# Autodesk Inventor assembly: HTPA32S2M100-A-P5
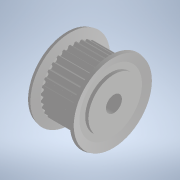
[picture p0: Inventor's stored thumbnail of the model, 180x180]
Saved by Autodesk Inventor 2021 (Build 250183000, 183)
## iProperties
Category: PARTsolutions
Company: MISUMI
Created: 2025-06-07
Part Number: HTPA32S2M100-A-P5
Catalog Web Link: www.cadenas.de
Description: HTPA_ _S2M040, HTPA_ _S2M060, HTPA_ _S2M100, HTPB_ _S2M040, HTPB_ _S2M060, HTPB_ _S2M100, HTPK_ _S2M040, HTPK_ _S2M060, HTPK_ _S2M100, HTPN_ _S2M040, HTPN_ _S2M060, HTPN_ _S2M100, HTPT_ _S2M040, HTPT_ _S2M060, HTPM_ _S2M040, HTPM_ _S2M060, HTPP_ _S2M040, HTPP_ _S2M060, HTPS_ _S2M040, HTPS_ _S2M060, HTPS_ _S2M100-High Torque Timing Pulleys S2M Type
Vendor: MISUMI
Document SubType Name: Assembly
Designer: psAdmin
Manufacturer: MISUMI
Mass: 4.1898 g
Surface Area: 29.6622 cm^2
Volume: 4.1898 cm^3
Density: 1 g/cm^3
Title: HTPA32S2M100-A-P5
Author: Cadenas PARTsolutions
Comments: High Torque Timing Pulleys S2M Type
PSOL_IDENT_0: {$CADENAS_DATA/23d-libs/misumi/metric/51_timing_pulleys/htpm_s2m_asmtab.prj},745 {VTYP=3D},{STYP=ASS
PSOL_IDENT_1: TAB},{NB=HTPA32S2M100-A-P5},{LINA=HTPA32S2M100-A-P5},{NN=HTPA_ _S2M040, HTPA_ _S2M060, HTPA_ _S2M100
PSOL_IDENT_2: , HTPB_ _S2M040, HTPB_ _S2M060, HTPB_ _S2M100, HTPK_ _S2M040, HTPK_ _S2M060, HTPK_ _S2M100, HTPN_ _S
PSOL_IDENT_3: 2M040, HTPN_ _S2M060, HTPN_ _S2M100, HTPT_ _S2M040, HTPT_ _S2M060, HTPM_ _S2M040, HTPM_ _S2M060, HTP
PSOL_IDENT_4: P_ _S2M040, HTPP_ _S2M060, HTPS_ _S2M040, HTPS_ _S2M060, HTPS_ _S2M100},{DATE=13.01.2023 00:39:47},{
PSOL_IDENT_5: GEOMDATE=09.12.2022 07:33:44},{VERSION=},{LINEID=170},{WBVAR=MATP,ST,TNW,PS,SBS,DD,Z,J,Q,R,S,T,ALT1,
PSOL_IDENT_6: ALT2,M,QSC,QFC,QTC,ALT3,K,KSC,KFC,KTC,ALT4,ZM,ZSC,ZFC,ZTC,ALT5,ALT6,ALT7,FC,ALT8,SRG,ALT9,BTC,TL,ALT
PSOL_IDENT_7: 10,TPC,ALT11,BC,ALT12,SLH,ALT13,BN},{WBNUMERIC=DD,Z,J,Q,R,S,T,QSC,QFC,QTC,K,KSC,KFC,KTC,ZSC,ZFC,ZTC,
PSOL_IDENT_8: FC,SRG,BTC,TL,BC,SLH,BN}  {NB=HTPA32S2M100-A-P5},{LINA=HTPA32S2M100-A-P5},{KT=DUMMY},{PN=HTPA32S2M10
PSOL_IDENT_9: 0-A-P5},{TYPE=HTPA},{MATP=A2017},{MATPALG= 'A2017','Aluminum Alloy 2000 series','S45CE','1045 Carbon
PSOL_IDENT_10: Steel Equivalent','SUS304','304 Stainless Steel' },{ST=CA},{STALG= 'CA' , 'Clear Anodize', 'BA','Bl
PSOL_IDENT_11: ack Anodize','HAT','Hard Clear Anodize' , 'ENP' , 'Electroless Nickel Plating' },{NT=32},{TNW=S2M100
PSOL_IDENT_12: },{TNWALG= 'S2M040', 'S2M060','S2M100' },{BW=10},{PS=A},{PSALG='A','B'},{SBS=P},{SBSALG= 'H','Round
PSOL_IDENT_13: Hole','P','Round Hole + Tap','N','New JIS Keywayed Bore + Tap (Standard)','V','Stepped Hole','Y','Bo
PSOL_IDENT_14: th Ends Stepped Hole','WB','Double Stepped Hole' },{SHSA= 'H','Round Hole','P','Round Hole + Tap','N'
PSOL_IDENT_15: ,'New JIS Keywayed Bore + Tap (Standard)','V','Stepped Hole','Y','Both Ends Stepped Hole','WB','Doub
PSOL_IDENT_16: le Stepped Hole' },{SHSB='H','Round Hole','P','Round Hole + Tap','V','Stepped Hole','F','Stepped Hol
PSOL_IDENT_17: e (Counterbore holes on the boss side)' },{SHSK='H','Round Hole','P','Round Hole + Tap'},{SBSPN=-P5}
PSOL_IDENT_18: ,{DD=5.00},{DDALG=[4:4/1],4.5,[5:6/1],6.35,[7:10/1]},{DDHA=[4:4/1],4.5,[5:6/1],6.35,[7:12/1]},{DDHBK=
PSOL_IDENT_19: 0},{DDPA=[4:4/1],4.5,[5:6/1],6.35,[7:10/1]},{DDPBK=0},{DDNA=[8:8/1]},{DDNBK=0},{DDNK=0},{DDCA=0},{DD
PSOL_IDENT_20: CBK=0},{DDVA=[4:4/1],4.5,[5:6/1],6.35,[7:10/1]},{DDVF=0},{DDY=[4:10/1]},{DDWB=[4:8/1]},{Z=0},{ZALG=[
PSOL_IDENT_21: 0]},{ZQRMIN=7},{ZAMAX=12},{ZBMAX=0},{DDZ=5},{J=0.0},{JALG=[0]},{JMAX=13},{JMIN=2},{JPN=},{QRMAX=12},
PSOL_IDENT_22: {QRMIN=7},{WBRMAX=-2.00},{WBQMIN=9},{Q=0},{QALG=[0]},{QPN=},{R=0},{RALG=[0]},{S=0.0},{SALG=[0]},{SPN=
PSOL_IDENT_23: },{SMAX=9},{T=0.0},{TALG=[0]},{TPN=},{TMAX=12},{A=11},{W=15},{L=0},{PD=20.37},{OD=19.86},{D=0},{DALG=
PSOL_IDENT_24: 12},{DE=16},{F=25},{E=16},{BBK=0.000},{TTK=0.0},{TT=1},{WL=15.000},{ALT1=},{ALT1ALG= '','w/o KC90 (S
PSOL_IDENT_25: et Screw Angle)','KC90','with KC90 (Set Screw Angle)' },{ANG=123.750},{ALT1PN=},{ALT2=},{ALT2ALG= ''
PSOL_IDENT_26: ,'Not applicable' },{M=N/A},{MALG= 'N/A' },{MFTALG= 'N/A' },{MSALG= 'N/A' },{M3D=0.000},{KDML=0},{ML=
PSOL_IDENT_27: 0},{MUL=0},{PITCH=0},{QSC=0.0},{QSCALG=0},{QFC=0.0},{QFCALG=0},{QTC=0.0},{QTCALG=0},{QPCDMIN=0},{QPC
PSOL_IDENT_28: DMINALG=0},{QPCDMAX=12},{ALT2PN=},{ALT3=},{ALT3ALG= '','Not applicable' },{K=0.0},{KALG=0},{KMIN=4},
PSOL_IDENT_29: {KFTMAX=0.0},{KSMAX=0.0},{KSC=0.0},{KSCALG=0},{KFC=0.0},{KFCALG=0},{KTC=0.0},{KTCALG=0},{KPCDMIN=9},
PSOL_IDENT_30: {KPCDMINALG=9},{KPCDMAX=12},{KSCMIN=9.0},{KSCMINALG=9},{ALT3PN=},{ALT4=},{ALT4ALG= '','Not applicabl
PSOL_IDENT_31: e' },{ALT4MIN=15.5},{ALT4MAX=5.5},{ZM=N/A},{ZMALG= 'N/A' },{ZMSALG= 'N/A' },{ZMFTALG= 'N/A' },{ZMDD1=
PSOL_IDENT_32: 0.0},{ZMDD2=0.0},{ZMHH=0.0},{ZSC=0.0},{ZSCALG=[0]},{ZFC=0.0},{ZFCALG=[0]},{ZTC=0.0},{ZTCALG=[0]},{ZP
PSOL_IDENT_33: CDMIN=0},{ZPCDMINALG=0},{ZPCDMAX=12},{ALT4PN=},{ALT5=},{ALT5ALG= '','Flange Attached','NFC','with NF
PSOL_IDENT_34: C (Flange not Attached)' },{ALT5PN=},{ALT6=},{ALT6ALG= '','w/o Flange Attached on One Side Only','RF
PSOL_IDENT_35: C','with RFC (Flange Attached on The Boss Side Only)','LFC','with LFC (Flange Attached on The Opposi
PSOL_IDENT_36: te Side Only)' },{ALT6PN=},{ALT7=},{ALT7ALG= '','w/o FC (Flange Cut)','FC','with FC (Flange Cut)' },
PSOL_IDENT_37: {FC=0.0},{FCALG=0},{FCMIN=21.0},{FCMAX=23.0},{ALT7PN=},{ALT8=},{ALT8ALG= '','Not applicable' },{ALT8
PSOL_IDENT_38: ALGALG=12},{ALT8DD2=0},{ALT8MM=0},{ALT8NN=0},{QC=0},{KC=0},{ZC=0},{SRG=0.0},{SRGALG=[0]},{SRGMAX=0},
PSOL_IDENT_39: {DD2=0.0},{MM=0.00},{NN=0.00},{ALT8PN=},{ALT9ALG= '','w/o BTC (Taper for Bearing Holder)','BTC','wit
PSOL_IDENT_40: h BTC (Taper for Bearing Holder)' },{ALT9=},{BTC9=7},{TL9=1},{BTC=0},{BTCALG=[0]},{TL=0.0},{TLALG=[0
PSOL_IDENT_41: ]},{TLMIN=1.000},{TLMAX=-15.500},{BTCL=0},{BTCD=0},{BTCDALG=12.000},{ALT9PN=},{WLBCTL=15},{ALT10=},{
PSOL_IDENT_42: ALT10ALG= '','w/o TPC (Tapped Hole Dimension)','TPC','with TPC (Tapped Hole Dimension)' },{TPC=N/A},
PSOL_IDENT_43: {TPCALG= 'N/A' },{TPCM=3},{ALT10PN=},{ALT11=},{ALT11ALG= '','Not applicable' },{BC=0.0},{BCALG=0},{B
PSOL_IDENT_44: CMIN=6},{BCMAX=-15.5},{BCPLANE=7.5},{M1WBC=7.5},{ALT11PN=},{ALT12=},{ALT12ALG= '','w/o SLH (Set Scre
PSOL_IDENT_45: w Length)','SLH','with SLH (Set Screw Length)' },{SLH=0},{SLHALG=[0]},{ALT12PN=},{ALT13=},{ALT13ALG=
PSOL_IDENT_46: '', 'Not applicable' },{BN=0.0},{BNALG=0},{BNMIN=-14.5},{BNMAX=-5},{ALT13PN=},{AC=M3x3},{M1=3},{M1L=
PSOL_IDENT_47: 3},{TAP=0.000},{KYY=2.5},{KTT=7.43},{PLANE=15},{PPATH=htpm_s2m/htpa_s2m_asmtpl.prj}
NB: HTPA32S2M100-A-P5
NN: 0
NT: 32
NBSYN: $PN.
LINA: HTPA32S2M100-A-P5
CATALOG: Misumi
PN: HTPA32S2M100-A-P5
MATP: Aluminum Alloy 2000 series
ST: Clear Anodize
TNW: S2M100
BW: 10
PS: A
SBS: Round Hole + Tap
DD: 5
Z: 0
J: 0
Q: 0
R: 0
S: 0
T: 0
A: 11
W: 15
L: 0
PD: 20.37
OD: 19.86
D: 0
F: 25
E: 16
TT: 1
ALT1: w/o KC90 (Set Screw Angle)
ALT2: Not applicable
M: N/A
QSC: 0
QFC: 0
QTC: 0
ALT3: Not applicable
K: 0
KSC: 0
KFC: 0
KTC: 0
ALT4: Not applicable
ZM: N/A
ZMDD1: 0
ZMDD2: 0
ZMHH: 0
ZSC: 0
ZFC: 0
ZTC: 0
ALT5: Flange Attached
ALT6: w/o Flange Attached on One Side Only
ALT7: w/o FC (Flange Cut)
FC: 0
ALT8: Not applicable
SRG: 0
DD2: 0
MM: 0
ALT9: w/o BTC (Taper for Bearing Holder)
BTC: 0
TL: 0
BTCL: 0
BTCD: 0
ALT10: w/o TPC (Tapped Hole Dimension)
TPC: N/A
ALT11: Not applicable
BC: 0
ALT12: w/o SLH (Set Screw Length)
SLH: 0
ALT13: Not applicable
BN: 0
AC: M3x3
SUPPLIER: MISUMI
ARTICLENO: HTPA32S2M100-A-P5
BOMINFO: HTPA32S2M100-A-P5
CREATOR: CADENAS GmbH
## Documents named in this file (3)
- e:\temp\worker_COMMON_293\temp\tmp_7720_2_IlNwC\format_0\HTPA32S2M100-A-P5.iam
- e:\temp\worker_COMMON_293\temp\tmp_7720_2_IlNwC\format_0\HTPA32S2M100-A-P5_a.ipt
- e:\temp\worker_COMMON_293\temp\tmp_7720_2_IlNwC\format_0\SET-SCREW3-3.ipt
## Components (3 placed, 2 different names)
1. HTPA32S2M100-A-P5_a:1 — to_s1_Z@1 <-> CP_Z@2, to_s2_Z@1 <-> CP_Z@3
2. SET-SCREW3-3:1 — to_s1_Z@1 <-> CP_Z@2
3. SET-SCREW3-3:2 — to_s2_Z@1 <-> CP_Z@3
## Relationships (2: Mate 2)
- to_s1_Z@1 <-> CP_Z@2 [Mate]: HTPA32S2M100-A-P5_a:1 ↔ SET-SCREW3-3:1
- to_s2_Z@1 <-> CP_Z@3 [Mate]: HTPA32S2M100-A-P5_a:1 ↔ SET-SCREW3-3:2
